# Autodesk Inventor assembly: Verbindungtuer
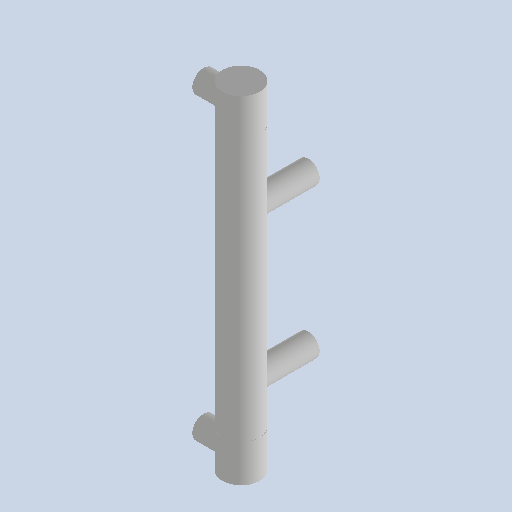
[picture p0: Inventor's stored thumbnail of the model, 512x512]
Saved by Autodesk Inventor 2025.1 (Build 291241000, 241)
## iProperties
Created: 2024-08-07
Part Number: Verbindungtuer
Document SubType Name: Assembly
Designer: ffogue
Author: ffogue
## Documents named in this file (3)
- C:\Users\ffogue\Documents\Inventor\BrandschutzTuer\Verbindungtuer.iam
- C:\Users\ffogue\Documents\Inventor\BrandschutzTuer\verbindung2.ipt
- C:\Users\ffogue\Documents\Inventor\BrandschutzTuer\verbindungoben.ipt
## Components (3 placed, 2 different names)
1. verbindung2:1 — Mate:1, Mate:2, Insert:1, Insert:2, Angle:1, Angle:2
2. verbindungoben:1 — Mate:1, Insert:1, Angle:2
3. verbindungoben:2 — Mate:2, Insert:2, Angle:1
## Relationships (6: Mate 2, Insert 2, Angle 2)
- Mate:1: verbindung2:1 ↔ verbindungoben:1
- Mate:2: verbindung2:1 ↔ verbindungoben:2
- Insert:1: verbindung2:1 ↔ verbindungoben:1
- Insert:2: verbindung2:1 ↔ verbindungoben:2
- Angle:1 (0 deg): verbindung2:1 ↔ verbindungoben:2
- Angle:2 (180 deg): verbindung2:1 ↔ verbindungoben:1
